# Autodesk Inventor assembly: mezzanineBoard
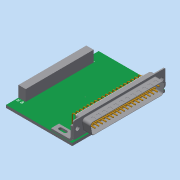
[picture p0: Inventor's stored thumbnail of the model, 180x180]
Saved by Autodesk Inventor 2016 (Build 200138000, 138)
## iProperties
Created: 2016-08-31
Part Number: mezzanineBoard
Document SubType Name: Assembly
Designer: Zara
Author: Zara
## Documents named in this file (5)
- C:\Users\Zara\Documents\hera-cad\Node\mezzanineBoard.iam
- C:\Users\Zara\Documents\hera-cad\Node\mezzaninePCB.ipt
- C:\Users\Zara\Documents\hera-cad\Node\snapPinout.ipt
- C:\Users\Zara\Documents\hera-cad\Node\173-E37-113.ipt
- C:\Users\Zara\Documents\hera-cad\Node\dsub37Bracket.ipt
## Components (5 placed, 4 different names)
1. mezzaninePCB:1 — Mate:2, Flush:3, Flush:4, Mate:4, Flush:5, Mate:5, Mate:8
2. snapPinout:1 — Mate:2, Flush:3, Flush:4
3. 173-E37-113:1 — Mate:4, Flush:5, Mate:6, Mate:7, Mate:9, Mate:10
4. dsub37Bracket:1 — Mate:5, Mate:6, Mate:7
5. dsub37Bracket:2 — Mate:8, Mate:9, Mate:10
## Relationships (11: Mate 8, Flush 3)
- Mate:2: mezzaninePCB:1 ↔ snapPinout:1
- Flush:3: mezzaninePCB:1 ↔ snapPinout:1
- Flush:4 (9.3 mm): mezzaninePCB:1 ↔ snapPinout:1
- Mate:4: mezzaninePCB:1 ↔ 173-E37-113:1
- Flush:5 (0.3556 mm): mezzaninePCB:1 ↔ 173-E37-113:1
- Mate:5: mezzaninePCB:1 ↔ dsub37Bracket:1
- Mate:6: 173-E37-113:1 ↔ dsub37Bracket:1
- Mate:7: 173-E37-113:1 ↔ dsub37Bracket:1
- Mate:8: mezzaninePCB:1 ↔ dsub37Bracket:2
- Mate:9: 173-E37-113:1 ↔ dsub37Bracket:2
- Mate:10: 173-E37-113:1 ↔ dsub37Bracket:2
